# Autodesk Inventor assembly: robot scrivi (2)
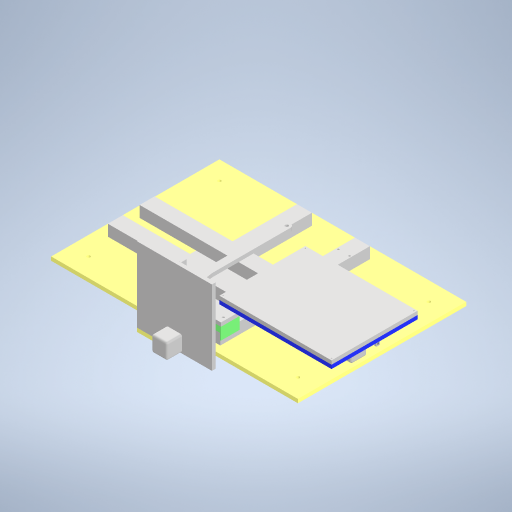
[picture p0: Inventor's stored thumbnail of the model, 512x512]
Saved by Autodesk Inventor 2024 (Build 280153000, 153)
## iProperties
Created: 2024-03-06
Part Number: robot scrivi (2)
Document SubType Name: Assembly
Designer: Giorgio
Author: Giorgio
## Documents named in this file (14)
- C:\Users\Giorgio\OneDrive\Desktop\me\inventor\pezzi robot scrivi\robot scrivi (2).iam
- C:\Users\Giorgio\OneDrive\Desktop\me\inventor\pezzi robot scrivi\base di lavoro.ipt
- C:\Users\Giorgio\OneDrive\Desktop\me\inventor\pezzi robot scrivi\cuscinetto.ipt
- C:\Users\Public\Documents\Autodesk\Inventor 2024\guida.ipt
- C:\Users\Giorgio\OneDrive\Desktop\me\inventor\pezzi robot scrivi\base sotto.ipt
- C:\Users\Giorgio\OneDrive\Desktop\me\inventor\pezzi robot scrivi\guide corte y.ipt
- C:\Users\Giorgio\OneDrive\Desktop\me\inventor\pezzi robot scrivi\base .ipt
- C:\Users\Giorgio\OneDrive\Desktop\me\inventor\pezzi robot scrivi\piano z.ipt
- C:\Users\Giorgio\OneDrive\Desktop\me\inventor\pezzi robot scrivi\guida z.ipt
- C:\Users\Giorgio\OneDrive\Desktop\me\inventor\pezzi robot scrivi\porta penna.ipt
- C:\Users\Giorgio\OneDrive\Desktop\me\inventor\pezzi robot scrivi\porta vite senza fine.ipt
- C:\Users\Giorgio\OneDrive\Desktop\me\inventor\pezzi robot scrivi\staffa motore.ipt
- C:\Users\Giorgio\OneDrive\Desktop\me\inventor\pezzi robot scrivi\motoreù.ipt
- C:\Users\Giorgio\OneDrive\Desktop\me\inventor\pezzi robot scrivi\base di lavoro sopra.ipt
## Components (25 placed, 13 different names)
1. base di lavoro:1 — Coincidente:32, Allineato:40, Allineato:41
2. cuscinetto:1 — Coincidente:30, Coincidente:31
3. cuscinetto:2
4. cuscinetto:3
5. cuscinetto:4
6. guida:1 — Allineato:38
7. guida:2 — Coincidente:30, Coincidente:31, Allineato:38, Allineato:39
8. base sotto:1 — Allineato:39
9. cuscinetto:5
10. cuscinetto:6
11. cuscinetto:7
12. cuscinetto:8
13. guide corte y:1
14. guide corte y:2
15. base :1
16. piano z:1
17. guida z:1
18. cuscinetto:9
19. porta penna:1
20. porta vite senza fine:1
21. porta vite senza fine:2
22. staffa motore:1
23. motoreù:1
24. motoreù:2
25. base di lavoro sopra:1 — Coincidente:32, Allineato:40, Allineato:41
## Relationships (69: Flush 38, Mate 31)
- [Mate] (-1 mm): base di lavoro:1 ↔ cuscinetto:1
- [Mate]: base di lavoro:1 ↔ cuscinetto:4
- [Mate]: base di lavoro:1 ↔ cuscinetto:2
- [Mate]: base di lavoro:1 ↔ cuscinetto:3
- [Flush]: cuscinetto:2 ↔ cuscinetto:4
- [Flush]: cuscinetto:1 ↔ cuscinetto:3
- [Flush]: cuscinetto:1 ↔ cuscinetto:4
- [Flush]: cuscinetto:2 ↔ cuscinetto:3
- [Flush] (-50 mm): base di lavoro:1 ↔ cuscinetto:3
- [Flush] (50 mm): base di lavoro:1 ↔ cuscinetto:3
- [Flush] (50 mm): base di lavoro:1 ↔ cuscinetto:2
- [Flush] (-50 mm): base di lavoro:1 ↔ cuscinetto:4
- [Mate]: cuscinetto:4 ↔ guida:1
- [Mate]: cuscinetto:4 ↔ guida:1
- [Mate]: guida:1 ↔ base sotto:1
- [Flush] (150 mm): guida:1 ↔ base sotto:1
- [Mate]: base sotto:1 ↔ cuscinetto:6
- [Mate]: base sotto:1 ↔ cuscinetto:5
- [Mate]: base sotto:1 ↔ cuscinetto:7
- [Mate]: base sotto:1 ↔ cuscinetto:8
- [Flush]: base sotto:1 ↔ cuscinetto:5
- [Flush]: cuscinetto:5 ↔ cuscinetto:6
- [Flush]: cuscinetto:5 ↔ cuscinetto:7
- [Flush]: base sotto:1 ↔ cuscinetto:5
- [Flush]: base sotto:1 ↔ cuscinetto:7
- [Flush]: base sotto:1 ↔ cuscinetto:6
- [Flush]: cuscinetto:6 ↔ cuscinetto:8
- [Flush]: cuscinetto:7 ↔ cuscinetto:8
- [Flush]: guide corte y:1 ↔ guide corte y:2
- [Flush]: guide corte y:1 ↔ guide corte y:2
- [Mate]: cuscinetto:5 ↔ guide corte y:1
- [Mate]: cuscinetto:7 ↔ guide corte y:1
- [Mate]: cuscinetto:8 ↔ guide corte y:2
- [Mate]: cuscinetto:8 ↔ guide corte y:2
- [Mate]: guide corte y:2 ↔ base :1
- [Flush] (237.5 mm): guide corte y:2 ↔ base :1
- [Flush] (-30 mm): guide corte y:2 ↔ base :1
- [Flush]: base :1 ↔ piano z:1
- [Mate] (-200 mm): base :1 ↔ piano z:1
- [Mate]: base :1 ↔ piano z:1
- [Mate]: piano z:1 ↔ guida z:1
- [Flush]: piano z:1 ↔ guida z:1
- [Flush] (92.55 mm): piano z:1 ↔ guida z:1
- [Mate]: guida z:1 ↔ cuscinetto:9
- [Mate]: guida z:1 ↔ cuscinetto:9
- [Mate]: cuscinetto:9 ↔ porta penna:1
- [Mate]: cuscinetto:9 ↔ porta penna:1
- [Flush]: cuscinetto:9 ↔ porta penna:1
- [Flush]: base di lavoro:1 ↔ porta vite senza fine:2
- [Mate]: base di lavoro:1 ↔ porta vite senza fine:2
- [Mate]: base sotto:1 ↔ porta vite senza fine:1
- [Flush]: base sotto:1 ↔ porta vite senza fine:1
- [Flush] (95 mm): base sotto:1 ↔ porta vite senza fine:1
- [Mate]: base sotto:1 ↔ staffa motore:1
- [Flush]: base sotto:1 ↔ staffa motore:1
- [Flush]: base sotto:1 ↔ staffa motore:1
- [Mate]: staffa motore:1 ↔ motoreù:1
- [Mate]: piano z:1 ↔ motoreù:2
- [Flush] (12 mm): base :1 ↔ motoreù:2
- [Flush] (80 mm): piano z:1 ↔ motoreù:2
- [Flush] (2 mm): staffa motore:1 ↔ motoreù:1
- [Flush] (4 mm): base sotto:1 ↔ motoreù:1
- Coincidente:30 [Mate]: cuscinetto:1 ↔ guida:2
- Coincidente:31 [Mate]: cuscinetto:1 ↔ guida:2
- Allineato:38 [Flush]: guida:1 ↔ guida:2
- Allineato:39 [Flush] (27.5 mm): guida:2 ↔ base sotto:1
- Coincidente:32 [Mate]: base di lavoro:1 ↔ base di lavoro sopra:1
- Allineato:40 [Flush]: base di lavoro:1 ↔ base di lavoro sopra:1
- Allineato:41 [Flush]: base di lavoro:1 ↔ base di lavoro sopra:1
## Named parameters: d11_d56 = 0 mm, d12_d57 = -200 mm, d13_d58 = 0 mm, d14_d61 = 0 mm, d15_d62 = 0 mm, d16_d63 = 92.55 mm, d17_d64 = 0 mm, d18_d65 = 0 mm, d19_d67 = 0 mm, d20_d68 = 0 mm, d21_d69 = 0 mm, d22_d30 = 0 mm, d23_d31 = 0 mm, d24_d32 = 0 mm, d25_d33 = 0 mm, d26_d34 = 0 mm, d27_d35 = 0 mm, d28_d36 = 0 mm, d29_d37 = 0 mm, d30_d38 = 0 mm, d31_d39 = 0 mm, d32_d40 = 0 mm, d33_d41 = 0 mm, d34_d43 = 0 mm, d35_d44 = 0 mm, d36_d45 = 0 mm, d37_d46 = 0 mm, d38_d47 = 0 mm, d39_d48 = 0 mm, d40_d50 = 0 mm, d41_d51 = 237.5 mm, d42_d52 = -30 mm
